# Autodesk Inventor assembly: WheelAssembly3.0
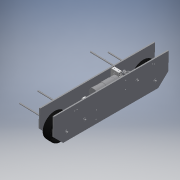
[picture p0: Inventor's stored thumbnail of the model, 180x180]
Saved by Autodesk Inventor 2017 (Build 210142000, 142)
## iProperties
Created: 2017-07-22
Part Number: WheelAssembly3.0
Document SubType Name: Assembly
Designer: User
Author: User
## Documents named in this file (15)
- C:\Robotics\CAD\2018-19_CAD\InvertedDriveTrain.iam
- C:\Robotics\CAD\COTSParts\Motors\Andymark 2964  NeveRest 40 Motor.ipt
- C:\Robotics\CAD\COTSParts\Tetrix\tetrix-motor-mounts-1.snapshot.1\Tetrex 2pc motor mount.ipt
- C:\Robotics\CAD\COTSParts\Actobotics\615 parts\615398.25inBoreBeveledGears.ipt
- C:\Robotics\CAD\2016-17_CAD\Custom COTS\4inax.ipt
- C:\Robotics\CAD\COTSParts\Actobotics\615 parts\615106Sprocket.5inBore.25inPitch24Teeth.ipt
- C:\Robotics\CAD\COTSParts\Actobotics\545 parts\545556SetScrewHub.77inPattern.ipt
- C:\Robotics\CAD\COTSParts\Wheels\4in Wheel Intergreated Hub 8mm Rev2.ipt
- C:\Robotics\CAD\2016-17_CAD\DriveTrain\MotorFixedPositionMount.ipt
- C:\Robotics\CAD\COTSParts\Actobotics\Thrust Bearings\6655K13.ipt
- C:\Robotics\CAD\2018-19_CAD\InvertedDrivePlateOutside.ipt
- C:\Robotics\CAD\2018-19_CAD\InvertedDrivePlateInside.ipt
- C:\Robotics\CAD\2018-19_CAD\Offseason\WheelandSprocketComboHub2.ipt
- C:\Robotics\CAD\COTSParts\Actobotics\535 parts\535198Bearing.25ID.5OD.ipt
- C:\Robotics\CAD\2018-19_CAD\Offseason\Tensioner3.iam
## Components (36 placed, 14 different names)
1. Andymark 2964  NeveRest 40 Motor:1 — Insert:3, Insert:6
2. Andymark 2964  NeveRest 40 Motor:2 — Insert:4, Insert:5
3. Tetrex 2pc motor mount:1 — Insert:3, Insert:48, Angle:7, Insert:79, Angle:8
4. Tetrex 2pc motor mount:2 — Insert:4, Insert:30, Angle:4, Insert:80, Angle:9
5. 615398.25inBoreBeveledGears:1 — Insert:5, Insert:44
6. 615398.25inBoreBeveledGears:2 — Insert:6, Insert:47
7. 615398.25inBoreBeveledGears:3 — Insert:77
8. 615398.25inBoreBeveledGears:4 — Insert:78
9. 4inax:1 — Insert:60, Mate:30
10. 4inax:2 — Insert:61
11. 615106Sprocket.5inBore.25inPitch24Teeth:2 — Insert:69, Flush:7
12. 4inax:3 — Insert:58, Mate:29
13. 4inax:4 — Insert:59
14. 545556SetScrewHub.77inPattern:4 — Insert:54
15. 4in Wheel Intergreated Hub 8mm Rev2:1 — Insert:65
16. 4in Wheel Intergreated Hub 8mm Rev2:2 — Insert:68
17. MotorFixedPositionMount:1 — Insert:30, Angle:4
18. MotorFixedPositionMount:2 — Insert:48, Angle:7
19. 545556SetScrewHub.77inPattern:7 — Insert:55
20. 615106Sprocket.5inBore.25inPitch24Teeth:3 — Insert:66, Flush:8
21. 6655K13:1 — Insert:64, Insert:78
22. 6655K13:2 — Insert:63, Insert:77
23. 6655K13:3 — Insert:44
24. 6655K13:4 — Insert:47
25. 615106Sprocket.5inBore.25inPitch24Teeth:4 — Insert:54, Mate:29, Flush:7
26. 615106Sprocket.5inBore.25inPitch24Teeth:5 — Insert:55, Mate:30, Flush:8
27. InvertedDrivePlateOutside:1 — Flush:1, Mate:24, Flush:2, Insert:58, Insert:59, Insert:60, Insert:61, Insert:71, Insert:72, Insert:73, Insert:74, Insert:75, Insert:76, Angle:10, Insert:81, Insert:82, Insert:83
28. InvertedDrivePlateInside:1 — Flush:1, Mate:24, Flush:2, Insert:63, Insert:64, Insert:79, Angle:8, Insert:80, Angle:9
29. WheelandSprocketComboHub2:1 — Insert:68, Insert:69, Insert:75
30. WheelandSprocketComboHub2:2 — Insert:65, Insert:66, Insert:76
31. 535198Bearing.25ID.5OD:1 — Insert:71
32. 535198Bearing.25ID.5OD:2 — Insert:74
33. 535198Bearing.25ID.5OD:3 — Insert:73
34. 535198Bearing.25ID.5OD:4 — Insert:72
35. Tensioner3:1 [sub-assembly] — Insert:82, Insert:83
36. Tensioner3:2 [sub-assembly] — Angle:10, Insert:81
## Relationships (45: Insert 33, Angle 5, Flush 4, Mate 3)
- Insert:3: Andymark 2964  NeveRest 40 Motor:1 ↔ Tetrex 2pc motor mount:1
- Insert:4: Andymark 2964  NeveRest 40 Motor:2 ↔ Tetrex 2pc motor mount:2
- Insert:5: Andymark 2964  NeveRest 40 Motor:2 ↔ 615398.25inBoreBeveledGears:1
- Insert:6: Andymark 2964  NeveRest 40 Motor:1 ↔ 615398.25inBoreBeveledGears:2
- Insert:30: Tetrex 2pc motor mount:2 ↔ MotorFixedPositionMount:1
- Insert:44: 615398.25inBoreBeveledGears:1 ↔ 6655K13:3
- Insert:47: 615398.25inBoreBeveledGears:2 ↔ 6655K13:4
- Insert:48: Tetrex 2pc motor mount:1 ↔ MotorFixedPositionMount:2
- Angle:4 (0 deg): Tetrex 2pc motor mount:2 ↔ MotorFixedPositionMount:1
- Insert:54: 545556SetScrewHub.77inPattern:4 ↔ 615106Sprocket.5inBore.25inPitch24Teeth:4
- Insert:55: 545556SetScrewHub.77inPattern:7 ↔ 615106Sprocket.5inBore.25inPitch24Teeth:5
- Angle:7 (0 deg): Tetrex 2pc motor mount:1 ↔ MotorFixedPositionMount:2
- Flush:1: InvertedDrivePlateOutside:1 ↔ InvertedDrivePlateInside:1
- Mate:24 (48.387 mm): InvertedDrivePlateOutside:1 ↔ InvertedDrivePlateInside:1
- Flush:2: InvertedDrivePlateOutside:1 ↔ InvertedDrivePlateInside:1
- Insert:58 (-6.35 mm): 4inax:3 ↔ InvertedDrivePlateOutside:1
- Insert:59 (-6.35 mm): 4inax:4 ↔ InvertedDrivePlateOutside:1
- Insert:60 (-6.35 mm): 4inax:1 ↔ InvertedDrivePlateOutside:1
- Insert:61 (-6.35 mm): 4inax:2 ↔ InvertedDrivePlateOutside:1
- Insert:63 (1.4224 mm): 6655K13:2 ↔ InvertedDrivePlateInside:1
- Insert:64 (-1.4224 mm): 6655K13:1 ↔ InvertedDrivePlateInside:1
- Insert:65: 4in Wheel Intergreated Hub 8mm Rev2:1 ↔ WheelandSprocketComboHub2:2
- Insert:66: 615106Sprocket.5inBore.25inPitch24Teeth:3 ↔ WheelandSprocketComboHub2:2
- Insert:68: 4in Wheel Intergreated Hub 8mm Rev2:2 ↔ WheelandSprocketComboHub2:1
- Insert:69: 615106Sprocket.5inBore.25inPitch24Teeth:2 ↔ WheelandSprocketComboHub2:1
- Insert:71: InvertedDrivePlateOutside:1 ↔ 535198Bearing.25ID.5OD:1
- Insert:72: InvertedDrivePlateOutside:1 ↔ 535198Bearing.25ID.5OD:4
- Insert:73: InvertedDrivePlateOutside:1 ↔ 535198Bearing.25ID.5OD:3
- Insert:74: InvertedDrivePlateOutside:1 ↔ 535198Bearing.25ID.5OD:2
- Insert:75 (1.27 mm): InvertedDrivePlateOutside:1 ↔ WheelandSprocketComboHub2:1
- Insert:76 (1.27 mm): InvertedDrivePlateOutside:1 ↔ WheelandSprocketComboHub2:2
- Insert:77: 615398.25inBoreBeveledGears:3 ↔ 6655K13:2
- Mate:29: 4inax:3 ↔ 615106Sprocket.5inBore.25inPitch24Teeth:4
- Flush:7: 615106Sprocket.5inBore.25inPitch24Teeth:2 ↔ 615106Sprocket.5inBore.25inPitch24Teeth:4
- Insert:78: 615398.25inBoreBeveledGears:4 ↔ 6655K13:1
- Mate:30: 4inax:1 ↔ 615106Sprocket.5inBore.25inPitch24Teeth:5
- Flush:8: 615106Sprocket.5inBore.25inPitch24Teeth:3 ↔ 615106Sprocket.5inBore.25inPitch24Teeth:5
- Insert:79: Tetrex 2pc motor mount:1 ↔ InvertedDrivePlateInside:1
- Angle:8 (0 deg): Tetrex 2pc motor mount:1 ↔ InvertedDrivePlateInside:1
- Insert:80: Tetrex 2pc motor mount:2 ↔ InvertedDrivePlateInside:1
- Angle:9 (0 deg): Tetrex 2pc motor mount:2 ↔ InvertedDrivePlateInside:1
- Angle:10 (-62 deg): InvertedDrivePlateOutside:1 ↔ Tensioner3:2
- Insert:81: InvertedDrivePlateOutside:1 ↔ Tensioner3:2
- Insert:82: InvertedDrivePlateOutside:1 ↔ Tensioner3:1
- Insert:83: InvertedDrivePlateOutside:1 ↔ Tensioner3:1
